# Autodesk Inventor assembly: POWER
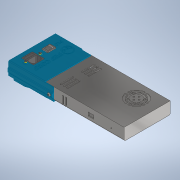
[picture p0: Inventor's stored thumbnail of the model, 180x180]
Saved by Autodesk Inventor 2020 (Build 240168000, 168)
## iProperties
Created: 2019-09-17
Part Number: POWER
Document SubType Name: Assembly
Designer: pepd9
Author: pepd9
## Documents named in this file (8)
- C:\DESIGNS\MK3PRO P1\PSU\POWER.iam
- C:\DESIGNS\MK3PRO P1\PSU\Mean Well LRS-350 Power Supply.ipt
- C:\DESIGNS\MK3PRO P1\COMPONENTS\BHCS M4x8.ipt
- C:\DESIGNS\MK3PRO P1\PSU\PSU COVER.ipt
- C:\DESIGNS\MK3PRO P1\PSU\IEC Receptacle.ipt
- C:\DESIGNS\MK3PRO P1\PSU\Rocker Switch.ipt
- C:\DESIGNS\MK3PRO P1\COMPONENTS\M3 Nut.ipt
- C:\DESIGNS\MK3PRO P1\COMPONENTS\SHCS_M3_10.ipt
## Components (13 placed, 7 different names)
1. Mean Well LRS-350 Power Supply:1 — Mate:1, Mate:2, Mate:3, Mate:4, Mate:5, Mate:30, Mate:31, Flush:1, Flush:2
2. BHCS M4x8:1 — Mate:2, Mate:3
3. BHCS M4x8:2 — Mate:1, Mate:4
4. PSU COVER:1 — Mate:5, Mate:8, Mate:11, Mate:12, Mate:13, Mate:14, Mate:15, Mate:16, Mate:17, Mate:18, Mate:19, Mate:20, Mate:21, Mate:22, Mate:23, Mate:24, Mate:25, Mate:26, Mate:27, Mate:28, Mate:29, Mate:30, Mate:31, Mate:32, Mate:33, Mate:34
5. BHCS M4x8:3 — Mate:8, Mate:13
6. BHCS M4x8:4 — Mate:12, Mate:33
7. BHCS M4x8:5 — Mate:11, Mate:32
8. IEC Receptacle:1 — Mate:14, Mate:15, Mate:16
9. Rocker Switch:1 — Mate:17, Mate:18, Mate:19
10. M3 Nut:1 — Mate:21, Mate:22, Mate:25
11. M3 Nut:2 — Mate:20, Mate:23, Mate:24
12. SHCS_M3_10:1 — Mate:27, Mate:28
13. SHCS_M3_10:2 — Mate:26, Mate:29
## Relationships (32: Mate 30, Flush 2)
- Mate:1: Mean Well LRS-350 Power Supply:1 ↔ BHCS M4x8:2
- Mate:2: Mean Well LRS-350 Power Supply:1 ↔ BHCS M4x8:1
- Mate:3 (6.35 mm): Mean Well LRS-350 Power Supply:1 ↔ BHCS M4x8:1
- Mate:4 (6.35 mm): Mean Well LRS-350 Power Supply:1 ↔ BHCS M4x8:2
- Mate:5: Mean Well LRS-350 Power Supply:1 ↔ PSU COVER:1
- Mate:8: PSU COVER:1 ↔ BHCS M4x8:3
- Mate:11: PSU COVER:1 ↔ BHCS M4x8:5
- Mate:12: PSU COVER:1 ↔ BHCS M4x8:4
- Mate:13: PSU COVER:1 ↔ BHCS M4x8:3
- Mate:14: PSU COVER:1 ↔ IEC Receptacle:1
- Mate:15: PSU COVER:1 ↔ IEC Receptacle:1
- Mate:16: PSU COVER:1 ↔ IEC Receptacle:1
- Mate:17: PSU COVER:1 ↔ Rocker Switch:1
- Mate:18: PSU COVER:1 ↔ Rocker Switch:1
- Mate:19: PSU COVER:1 ↔ Rocker Switch:1
- Mate:20: PSU COVER:1 ↔ M3 Nut:2
- Mate:21: PSU COVER:1 ↔ M3 Nut:1
- Mate:22: PSU COVER:1 ↔ M3 Nut:1
- Mate:23: PSU COVER:1 ↔ M3 Nut:2
- Mate:24: PSU COVER:1 ↔ M3 Nut:2
- Mate:25: PSU COVER:1 ↔ M3 Nut:1
- Mate:26: PSU COVER:1 ↔ SHCS_M3_10:2
- Mate:27: PSU COVER:1 ↔ SHCS_M3_10:1
- Mate:28: PSU COVER:1 ↔ SHCS_M3_10:1
- Mate:29: PSU COVER:1 ↔ SHCS_M3_10:2
- Mate:30: Mean Well LRS-350 Power Supply:1 ↔ PSU COVER:1
- Mate:31: Mean Well LRS-350 Power Supply:1 ↔ PSU COVER:1
- Mate:32: PSU COVER:1 ↔ BHCS M4x8:5
- Mate:33: PSU COVER:1 ↔ BHCS M4x8:4
- Flush:1: Mean Well LRS-350 Power Supply:1
- Flush:2: Mean Well LRS-350 Power Supply:1
- Mate:34: PSU COVER:1
